# Autodesk Inventor assembly: ExtendedServoPlateProjected
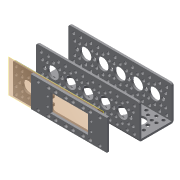
[picture p0: Inventor's stored thumbnail of the model, 180x180]
Saved by Autodesk Inventor 2018 (Build 220112000, 112)
## iProperties
Created: 2018-12-08
Part Number: ExtendedServoPlateProjected
Document SubType Name: Assembly
Designer: ball
Author: ball
## Documents named in this file (4)
- C:\FTC\FTC8863CAD\2018Robot\ExtendedServoPlateProjected.iam
- C:\FTC\FTC8863CAD\Actobotics\575 parts\575144.ipt
- C:\FTC\FTC8863CAD\Actobotics\585 parts\585444.ipt
- C:\FTC\FTC8863CAD\2018Robot\ExtendedServoMount.ipt
## Components (3 placed, 3 different names)
1. 575144:1 — Mate:1, Mate:2, Mate:3, Flush:1, Flush:2
2. 585444:1 — Mate:1, Mate:2, Mate:3
3. ExtendedServoMount:1 — Flush:1, Flush:2
## Relationships (5: Mate 3, Flush 2)
- Mate:1 (25.4 mm): 575144:1 ↔ 585444:1
- Mate:2: 575144:1 ↔ 585444:1
- Mate:3: 575144:1 ↔ 585444:1
- Flush:1: 575144:1 ↔ ExtendedServoMount:1
- Flush:2: 575144:1 ↔ ExtendedServoMount:1
